# Autodesk Inventor assembly: EM Plate
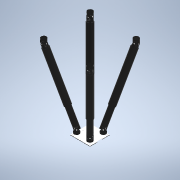
[picture p0: Inventor's stored thumbnail of the model, 180x180]
Saved by Autodesk Inventor 2022 (Build 260153000, 153)
## iProperties
Created: 2022-02-15
Part Number: EM Plate
Document SubType Name: Assembly
Designer: RNG3nius
Author: RNG3nius
## Documents named in this file (8)
- C:\Users\Dahway\Documents\GitHub\GMU-RobotX-Mechanical\Object Retrieval\V1\EM Plate.iam
- C:\Users\Dahway\Documents\GitHub\GMU-RobotX-Mechanical\Object Retrieval\V1\EM plate.ipt
- C:\Users\Dahway\Documents\GitHub\GMU-RobotX-Mechanical\Object Retrieval\V1\joint.ipt
- C:\Users\Dahway\Documents\GitHub\GMU-RobotX-Mechanical\Object Retrieval\V1\Nut.ipt
- C:\Users\Dahway\Documents\GitHub\GMU-RobotX-Mechanical\Object Retrieval\V1\shaft.ipt
- C:\Users\Dahway\Documents\GitHub\GMU-RobotX-Mechanical\Object Retrieval\V1\inner tube.ipt
- C:\Users\Dahway\Documents\GitHub\GMU-RobotX-Mechanical\Object Retrieval\V1\outer tube.ipt
- C:\Users\Dahway\Documents\GitHub\GMU-RobotX-Mechanical\Object Retrieval\V1\magnet.ipt
## Components (66 placed, 7 different names)
1. EM plate:1 — Mate:1, Mate:2, Mate:13, Mate:14, Angle:1
2. magnet:1 — Mate:13, Mate:14
3. joint:1 — Mate:1, Mate:2
4. joint:2
5. joint:3 — Rotation:1, Rotational:1
6. joint:4
7. Nut:1 — Mate:15, Mate:16
8. joint:5 — Rigid:1, Mate:17, Mate:18
9. inner tube:1 — Mate:17, Mate:18, Mate:19, Mate:20
10. outer tube:1 — Mate:19, Mate:20, Mate:21, Mate:22
11. joint:6 — Mate:21, Mate:22, Rotational:2
12. Nut:2 — Mate:23, Mate:24
13. joint:7 — Rotational:3, Angle:1
14. Nut:3
15. joint:8
16. inner tube:2
17. outer tube:2
18. joint:9
19. Nut:4
20. joint:10
21. Nut:5
22. joint:11
23. inner tube:3
24. outer tube:3
25. joint:12
26. Nut:6
27. joint:13
28. Nut:7
29. joint:14
30. inner tube:4
31. outer tube:4
32. joint:15
33. Nut:8
34. joint:16
35. shaft:1 — Mate:15, Mate:16, Rigid:1
36. shaft:2 — Rotation:1, Rotational:1
37. shaft:3
38. shaft:4
39. shaft:5 — Mate:23, Mate:24
40. shaft:6 — Rotational:2
41. shaft:7 — Rotational:3
42. shaft:8
43. shaft:9
44. shaft:10
45. shaft:11
46. shaft:12
47. shaft:13
48. shaft:14
49. shaft:15
50. shaft:16
51. shaft:17
52. shaft:18
53. shaft:19
54. shaft:20
55. shaft:21
56. shaft:22
57. shaft:23
58. shaft:24
59. shaft:25
60. shaft:26
61. shaft:27
62. shaft:28
63. shaft:29
64. shaft:30
65. shaft:31
66. shaft:32
## Component patterns: (4 elements, first: joint:1), (4 elements, first: Nut:1 + joint:5 + inner tube:1 + outer tube:1 + joint:6 + Nut:2 + joint:7), (4 elements, first: shaft:1), (4 elements, first: shaft:5), Component Pattern 6:2 (4 elements), Component Pattern 7:2 (4 elements), Component Pattern 6:3 (4 elements), Component Pattern 7:3 (4 elements), Component Pattern 6:4 (4 elements), Component Pattern 7:4 (4 elements)
## Relationships (20: Mate 14, RevoluteJoint 3, RelateRotation 1, WeldJoint 1, Angle 1)
- Mate:1: EM plate:1 ↔ joint:1
- Mate:2: EM plate:1 ↔ joint:1
- Mate:13: EM plate:1 ↔ magnet:1
- Mate:14: EM plate:1 ↔ magnet:1
- Mate:15: Nut:1 ↔ shaft:1
- Mate:16: Nut:1 ↔ shaft:1
- Rotation:1 [RelateRotation] (1 ul): joint:3 ↔ shaft:2
- Rotational:1 [RevoluteJoint]: joint:3 ↔ shaft:2
- Rigid:1 [WeldJoint]: joint:5 ↔ shaft:1
- Mate:17: joint:5 ↔ inner tube:1
- Mate:18: joint:5 ↔ inner tube:1
- Mate:19: inner tube:1 ↔ outer tube:1
- Mate:20: inner tube:1 ↔ outer tube:1
- Mate:21: outer tube:1 ↔ joint:6
- Mate:22: outer tube:1 ↔ joint:6
- Mate:23: Nut:2 ↔ shaft:5
- Mate:24: Nut:2 ↔ shaft:5
- Rotational:2 [RevoluteJoint]: joint:6 ↔ shaft:6
- Rotational:3 [RevoluteJoint]: joint:7 ↔ shaft:7
- Angle:1 (0 deg): EM plate:1 ↔ joint:7
